# Autodesk Inventor assembly: 前腕_1
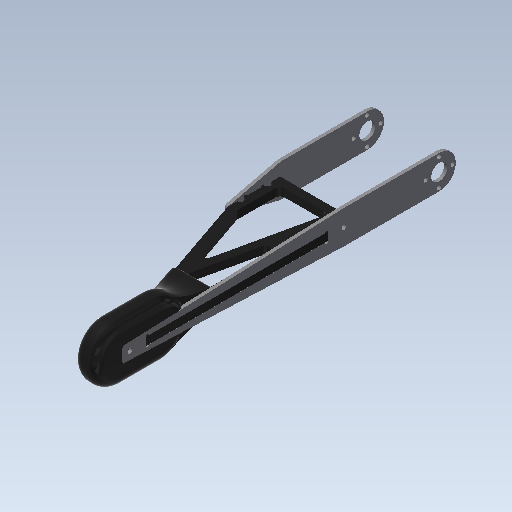
[picture p0: Inventor's stored thumbnail of the model, 512x512]
Saved by Autodesk Inventor 2020.3 (Build 243373000, 373)
## iProperties
Created: 2016-05-04
Part Number: 前腕_1
Document SubType Name: Assembly
Designer: hiroaki
Mass: 59.7567 g
Surface Area: 275.043 cm^2
Volume: 46.6042 cm^3
Density: 1.28222 g/cm^3
Author: hiroaki
## Documents named in this file (5)
- C:\Users\masato\Documents\Inventor\CITBrains\スパイク\OpenPlatform_ver3_0\上半身\腕\前腕_1.iam
- C:\Users\masato\Documents\Inventor\CITBrains\スパイク\OpenPlatform_ver3_0\上半身\腕\前腕_メインフレーム_1_1.ipt
- C:\Users\masato\Documents\Inventor\CITBrains\スパイク\OpenPlatform_ver3_0\上半身\腕\前腕_サブフレーム_1_1.ipt
- C:\Users\masato\Documents\Inventor\CITBrains\スパイク\OpenPlatform_ver3_0\上半身\腕\前腕_メインフレーム_1_2.ipt
- C:\Users\masato\Documents\Inventor\CITBrains\スパイク\OpenPlatform_ver3_0\上半身\腕\腕先.ipt
## Components (4 placed, 4 different names)
1. 前腕_メインフレーム_1_1:1 — 挿入:3, 挿入:4, メイト:3
2. 前腕_サブフレーム_1_1:1 — メイト:1, メイト:2, フラッシュ:1, 挿入:3, 挿入:4, 挿入:5, 挿入:6, メイト:5, メイト:6
3. 前腕_メインフレーム_1_2:1 — 挿入:5, 挿入:6
4. 腕先:1 — メイト:3, メイト:5, メイト:6
## Relationships (10: Mate 5, Insert 4, Flush 1)
- メイト:1 [Mate]: 前腕_サブフレーム_1_1:1
- メイト:2 [Mate]: 前腕_サブフレーム_1_1:1
- フラッシュ:1 [Flush]: 前腕_サブフレーム_1_1:1
- 挿入:3 [Insert]: 前腕_メインフレーム_1_1:1 ↔ 前腕_サブフレーム_1_1:1
- 挿入:4 [Insert]: 前腕_メインフレーム_1_1:1 ↔ 前腕_サブフレーム_1_1:1
- 挿入:5 [Insert]: 前腕_サブフレーム_1_1:1 ↔ 前腕_メインフレーム_1_2:1
- 挿入:6 [Insert]: 前腕_サブフレーム_1_1:1 ↔ 前腕_メインフレーム_1_2:1
- メイト:3 [Mate]: 前腕_メインフレーム_1_1:1 ↔ 腕先:1
- メイト:5 [Mate]: 前腕_サブフレーム_1_1:1 ↔ 腕先:1
- メイト:6 [Mate]: 前腕_サブフレーム_1_1:1 ↔ 腕先:1
